# Autodesk Inventor assembly: Y_GANTRY
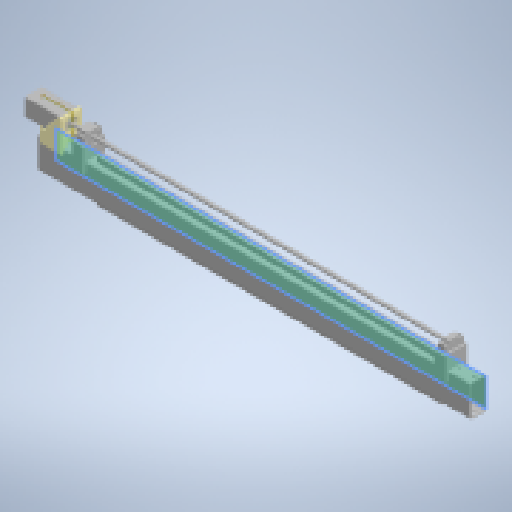
[picture p0: Inventor's stored thumbnail of the model, 512x512]
Saved by Autodesk Inventor 2023 (Build 270158000, 158)
## iProperties
Created: 2023-06-21
Part Number: Y_GANTRY
Document SubType Name: Assembly
Designer: plebbb
Author: plebbb
## Documents named in this file (11)
- D:\Users\plebbb\Desktop\CNC_Project\Y_GANTRY.iam
- D:\Users\plebbb\Desktop\CNC_Project\2x4_Tube.ipt
- D:\Users\plebbb\Desktop\CNC_Project\HGW20CC_Rail_800mm.ipt
- D:\Users\plebbb\Desktop\CNC_Project\BK10.ipt
- D:\Users\plebbb\Desktop\CNC_Project\BF10.ipt
- D:\Users\plebbb\Desktop\CNC_Project\SFU1204-500.ipt
- D:\Users\plebbb\Desktop\CNC_Project\BF10_Spacer.ipt
- D:\Users\plebbb\Desktop\CNC_Project\BK10_Spacer.ipt
- D:\Users\plebbb\Desktop\CNC_Project\Nema23.ipt
- D:\Users\plebbb\Desktop\CNC_Project\Nema23_Mount_short.ipt
- D:\Users\plebbb\Desktop\CNC_Project\2x4_Endcap.ipt
## Components (11 placed, 10 different names)
1. 2x4_Tube:1 — Mate:21, Mate:22, Mate:23
2. HGW20CC_Rail_800mm:1
3. BK10:1
4. BF10:1
5. SFU1204-500:1
6. BF10_Spacer:1
7. BK10_Spacer:1
8. HGW20CC_Rail_800mm:2
9. Nema23:1
10. Nema23_Mount_short:1
11. 2x4_Endcap:1 — Mate:21, Mate:22, Mate:23
## Relationships (27: Mate 23, Flush 4)
- [Flush] (15.4 mm): 2x4_Tube:1 ↔ HGW20CC_Rail_800mm:1
- [Mate]: 2x4_Tube:1 ↔ HGW20CC_Rail_800mm:1
- [Mate]: 2x4_Tube:1 ↔ BK10_Spacer:1
- [Mate]: 2x4_Tube:1 ↔ BK10_Spacer:1
- [Mate]: BF10:1 ↔ BF10_Spacer:1
- [Mate]: BF10:1 ↔ BF10_Spacer:1
- [Mate]: BF10:1 ↔ BF10_Spacer:1
- [Mate]: 2x4_Tube:1 ↔ BF10_Spacer:1
- [Mate]: 2x4_Tube:1 ↔ BF10_Spacer:1
- [Mate]: BF10:1 ↔ SFU1204-500:1
- [Flush] (70 mm): 2x4_Tube:1 ↔ BF10_Spacer:1
- [Mate]: HGW20CC_Rail_800mm:1 ↔ BF10_Spacer:1
- [Mate]: BK10:1 ↔ BK10_Spacer:1
- [Mate]: BK10:1 ↔ BK10_Spacer:1
- [Mate]: BK10:1 ↔ BK10_Spacer:1
- [Mate]: BK10:1 ↔ SFU1204-500:1
- [Flush]: HGW20CC_Rail_800mm:1 ↔ HGW20CC_Rail_800mm:2
- [Mate]: 2x4_Tube:1 ↔ HGW20CC_Rail_800mm:2
- [Flush]: HGW20CC_Rail_800mm:1 ↔ HGW20CC_Rail_800mm:2
- [Mate]: 2x4_Tube:1 ↔ Nema23_Mount_short:1
- [Mate] (0.25 mm): 2x4_Tube:1 ↔ Nema23_Mount_short:1
- [Mate]: SFU1204-500:1 ↔ Nema23:1
- [Mate]: SFU1204-500:1 ↔ Nema23:1
- [Mate]: Nema23:1 ↔ Nema23_Mount_short:1
- Mate:21 (0.2 mm): 2x4_Tube:1 ↔ 2x4_Endcap:1
- Mate:22 (0.2 mm): 2x4_Tube:1 ↔ 2x4_Endcap:1
- Mate:23: 2x4_Tube:1 ↔ 2x4_Endcap:1
## Named parameters: d34_d67 = 0 mm, d6_d21 = 15.4 mm, d7_d22 = 0 mm
